# Autodesk Inventor assembly: WheelNChainGear
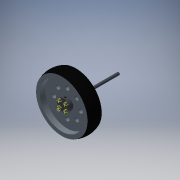
[picture p0: Inventor's stored thumbnail of the model, 180x180]
Saved by Autodesk Inventor 2016 (Build 200138000, 138)
## iProperties
Created: 2015-08-30
Part Number: WheelNChainGear
Document SubType Name: Assembly
Designer: Tim
Author: Tim
## Documents named in this file (7)
- C:\Users\Tim\Documents\GitHub\phi_robotics\3d-models\FTC_Tetrix_KOP_Block_Party\Tim Bloot Designs\WheelNChainGear.iam
- C:\Users\Tim\Documents\GitHub\phi_robotics\3d-models\FTC_Tetrix_KOP_Block_Party\Tetrix_Kit_FTC\Autodesk Inventor Files\tetrix_wheel.ipt
- C:\Users\Tim\Documents\GitHub\phi_robotics\3d-models\FTC_Tetrix_KOP_Block_Party\Tetrix_Kit_FTC\Autodesk Inventor Files\tetrix_axle_lock.iam
- C:\Users\Tim\Documents\GitHub\phi_robotics\3d-models\FTC_Tetrix_KOP_Block_Party\Tetrix_Kit_FTC\Autodesk Inventor Files\tetrix_axle_spacer_mount.ipt
- C:\Users\Tim\Documents\GitHub\phi_robotics\3d-models\FTC_Tetrix_KOP_Block_Party\Tetrix_Kit_FTC\Autodesk Inventor Files\tetrix_axle.ipt
- C:\Users\Tim\Documents\GitHub\phi_robotics\3d-models\FTC_Tetrix_KOP_Block_Party\Tetrix_Kit_FTC\Autodesk Inventor Files\tetrix_chain_gear-32t.ipt
- C:\Users\Tim\Documents\GitHub\phi_robotics\3d-models\FTC_Tetrix_KOP_Block_Party\Tetrix_Kit_FTC\Autodesk Inventor Files\tetrix_motor_screw-long.ipt
## Components (10 placed, 6 different names)
1. tetrix_wheel:1 — Rigid:1, Rigid:4
2. tetrix_axle_lock:1 [sub-assembly] — Rigid:4, Rigid:5, Rotational:1, Rotational:2, Rotational:3, Rotational:4
3. tetrix_axle_spacer_mount:1 — Rigid:1, Rigid:6
4. tetrix_axle:1 — Rigid:5
5. tetrix_chain_gear-32t:2 — Rigid:6, Rigid:7
6. tetrix_axle_lock:2 [sub-assembly] — Rigid:7
7. tetrix_motor_screw-long:1 — Rotational:1
8. tetrix_motor_screw-long:2 — Rotational:2
9. tetrix_motor_screw-long:3 — Rotational:4
10. tetrix_motor_screw-long:4 — Rotational:3
## Relationships (9: WeldJoint 5, RevoluteJoint 4)
- Rigid:1 [WeldJoint]: tetrix_wheel:1 ↔ tetrix_axle_spacer_mount:1
- Rigid:4 [WeldJoint]: tetrix_wheel:1 ↔ tetrix_axle_lock:1
- Rigid:5 [WeldJoint] (-1 mm): tetrix_axle_lock:1 ↔ tetrix_axle:1
- Rigid:6 [WeldJoint]: tetrix_axle_spacer_mount:1 ↔ tetrix_chain_gear-32t:2
- Rigid:7 [WeldJoint]: tetrix_chain_gear-32t:2 ↔ tetrix_axle_lock:2
- Rotational:1 [RevoluteJoint]: tetrix_axle_lock:1 ↔ tetrix_motor_screw-long:1
- Rotational:2 [RevoluteJoint]: tetrix_axle_lock:1 ↔ tetrix_motor_screw-long:2
- Rotational:3 [RevoluteJoint]: tetrix_axle_lock:1 ↔ tetrix_motor_screw-long:4
- Rotational:4 [RevoluteJoint]: tetrix_axle_lock:1 ↔ tetrix_motor_screw-long:3
